# Autodesk Inventor assembly: JGB37-520
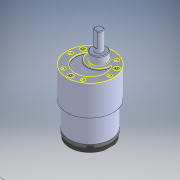
[picture p0: Inventor's stored thumbnail of the model, 180x180]
Saved by Autodesk Inventor 2022 (Build 260153000, 153)
## iProperties
Created: 2017-03-27
Part Number: JGB37-520
Description: STEP AP214
Document SubType Name: Assembly
Designer: Petrov Ivan
Sending System: SolidWorks 2017
Preprocessor: SwSTEP 2.0
Title: JGB37-520.STEP
Revision Number: ANY
## Documents named in this file (10)
- D:\IVAN\Ivan_desktop\Kvantorium\Projects\YouBotRobot\design\standart_components\JGB37-520\JGB37-520.iam
- D:\IVAN\Ivan_desktop\Kvantorium\Projects\YouBotRobot\design\standart_components\JGB37-520\GEARED BODY, MOTOR, JGB37-520.ipt
- D:\IVAN\Ivan_desktop\Kvantorium\Projects\YouBotRobot\design\standart_components\JGB37-520\DC MOTOR, JGB37-520.ipt
- D:\IVAN\Ivan_desktop\Kvantorium\Projects\YouBotRobot\design\standart_components\JGB37-520\MOTOR SHAFT, JGB37-520.ipt
- D:\IVAN\Ivan_desktop\Kvantorium\Projects\YouBotRobot\design\standart_components\JGB37-520\SHAFT COUPLER, JGB37-520.ipt
- D:\IVAN\Ivan_desktop\Kvantorium\Projects\YouBotRobot\design\standart_components\JGB37-520\COUPLING BRACKET, GEARED BODY TO DC MOTOR, JGB37-520.ipt
- D:\IVAN\Ivan_desktop\Kvantorium\Projects\YouBotRobot\design\standart_components\JGB37-520\PLASTIC COVER, DC MOTOR, JGB37-520.ipt
- D:\IVAN\Ivan_desktop\Kvantorium\Projects\YouBotRobot\design\standart_components\JGB37-520\CONNECTION, DC MOTOR, JGB37-520.ipt
- D:\IVAN\Ivan_desktop\Kvantorium\Projects\YouBotRobot\design\standart_components\JGB37-520\pan cross head_am_B18.6.7M - M2 x 0.4 x 25 Type I Cross Recessed PHMS --25N.ipt
- D:\IVAN\Ivan_desktop\Kvantorium\Projects\YouBotRobot\design\encoder.ipt
## Components (12 placed, 12 different names)
1. GEARED BODY, MOTOR, JGB37-520_1 — Заподлицо:1, Совмещение:3, Совмещение:5, Совмещение:6, Совмещение:7, Совмещение:8, Совмещение:12, Совмещение:13
2. DC MOTOR, JGB37-520_2 — Совмещение:1, Совмещение:3
3. MOTOR SHAFT, JGB37-520_3 — Совмещение:14, Совмещение:15
4. SHAFT COUPLER, JGB37-520_4 — Совмещение:12, Совмещение:13, Совмещение:14, Совмещение:15
5. COUPLING BRACKET, GEARED BODY TO DC MOTOR, JGB37-520_5 — Заподлицо:1, Совмещение:4, Совмещение:9, Совмещение:10, Совмещение:11
6. PLASTIC COVER, DC MOTOR, JGB37-520_6
7. CONNECTION, DC MOTOR, JGB37-520_7
8. CONNECTION, DC MOTOR, JGB37-520_8 — Совмещение:2, Угол:1
9. pan cross head_am_B18.6.7M - M2 x 0.4 x 25 Type I Cross Recessed PHMS --25N_9 — Совмещение:7, Совмещение:8, Совмещение:9
10. pan cross head_am_B18.6.7M - M2 x 0.4 x 25 Type I Cross Recessed PHMS --25N_10 — Совмещение:4, Совмещение:5, Совмещение:10
11. pan cross head_am_B18.6.7M - M2 x 0.4 x 25 Type I Cross Recessed PHMS --25N_11 — Совмещение:6, Совмещение:11
12. encoder:1 — Совмещение:1, Совмещение:2, Угол:1
## Relationships (17: Mate 15, Angle 1, Flush 1)
- Совмещение:1 [Mate]: DC MOTOR, JGB37-520_2 ↔ encoder:1
- Совмещение:2 [Mate]: CONNECTION, DC MOTOR, JGB37-520_8 ↔ encoder:1
- Угол:1 [Angle] (179.9087 deg): CONNECTION, DC MOTOR, JGB37-520_8 ↔ encoder:1
- Заподлицо:1 [Flush]: GEARED BODY, MOTOR, JGB37-520_1 ↔ COUPLING BRACKET, GEARED BODY TO DC MOTOR, JGB37-520_5
- Совмещение:3 [Mate]: GEARED BODY, MOTOR, JGB37-520_1 ↔ DC MOTOR, JGB37-520_2
- Совмещение:4 [Mate]: COUPLING BRACKET, GEARED BODY TO DC MOTOR, JGB37-520_5 ↔ pan cross head_am_B18.6.7M - M2 x 0.4 x 25 Type I Cross Recessed PHMS --25N_10
- Совмещение:5 [Mate]: GEARED BODY, MOTOR, JGB37-520_1 ↔ pan cross head_am_B18.6.7M - M2 x 0.4 x 25 Type I Cross Recessed PHMS --25N_10
- Совмещение:6 [Mate]: GEARED BODY, MOTOR, JGB37-520_1 ↔ pan cross head_am_B18.6.7M - M2 x 0.4 x 25 Type I Cross Recessed PHMS --25N_11
- Совмещение:7 [Mate]: GEARED BODY, MOTOR, JGB37-520_1 ↔ pan cross head_am_B18.6.7M - M2 x 0.4 x 25 Type I Cross Recessed PHMS --25N_9
- Совмещение:8 [Mate]: GEARED BODY, MOTOR, JGB37-520_1 ↔ pan cross head_am_B18.6.7M - M2 x 0.4 x 25 Type I Cross Recessed PHMS --25N_9
- Совмещение:9 [Mate]: COUPLING BRACKET, GEARED BODY TO DC MOTOR, JGB37-520_5 ↔ pan cross head_am_B18.6.7M - M2 x 0.4 x 25 Type I Cross Recessed PHMS --25N_9
- Совмещение:10 [Mate]: COUPLING BRACKET, GEARED BODY TO DC MOTOR, JGB37-520_5 ↔ pan cross head_am_B18.6.7M - M2 x 0.4 x 25 Type I Cross Recessed PHMS --25N_10
- Совмещение:11 [Mate]: COUPLING BRACKET, GEARED BODY TO DC MOTOR, JGB37-520_5 ↔ pan cross head_am_B18.6.7M - M2 x 0.4 x 25 Type I Cross Recessed PHMS --25N_11
- Совмещение:12 [Mate]: GEARED BODY, MOTOR, JGB37-520_1 ↔ SHAFT COUPLER, JGB37-520_4
- Совмещение:13 [Mate]: GEARED BODY, MOTOR, JGB37-520_1 ↔ SHAFT COUPLER, JGB37-520_4
- Совмещение:14 [Mate]: MOTOR SHAFT, JGB37-520_3 ↔ SHAFT COUPLER, JGB37-520_4
- Совмещение:15 [Mate] (-6.5 mm): MOTOR SHAFT, JGB37-520_3 ↔ SHAFT COUPLER, JGB37-520_4
